# Autodesk Inventor assembly: s-assy-sorter
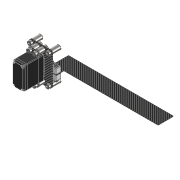
[picture p0: Inventor's stored thumbnail of the model, 180x180]
Saved by Autodesk Inventor 2022 (Build 260153000, 153)
## iProperties
Created: 2021-08-27
Part Number: s-assy-sorter
Document SubType Name: Assembly
Designer: Yuta Kage
Author: Yuta Kage
## Documents named in this file (9)
- C:\Users\yuta0\Documents\GitHub\catchrobo_hardware\assy-shooter\s-assy-sorter.iam
- C:\Users\yuta0\Documents\GitHub\catchrobo_hardware\assy-shooter\s-assy-shooter_motor.iam
- C:\Users\yuta0\Documents\GitHub\catchrobo_hardware\assy-shooter\s_base3.ipt
- C:\Users\yuta0\Documents\GitHub\catchrobo_hardware\assy-shooter\CB3-25.ipt
- C:\Users\yuta0\Documents\GitHub\catchrobo_hardware\assy-shooter\s_carbon_plate2.ipt
- C:\Users\yuta0\Documents\GitHub\catchrobo_hardware\assy-robot\CBSTNR3-12.ipt
- C:\Users\yuta0\Documents\GitHub\catchrobo_hardware\assy-robot\LBNR3.ipt
- C:\Users\yuta0\Documents\GitHub\catchrobo_hardware\assy-robot\ARF-415.ipt
- C:\Users\yuta0\Documents\GitHub\catchrobo_hardware\assy-robot\CB4-6.ipt
## Components (19 placed, 8 different names)
1. s-assy-shooter_motor:1 [sub-assembly] — メイト:6, メイト:7, メイト:12, メイト:13, メイト:14, メイト:15, メイト:16, メイト:17, メイト:18, メイト:19, メイト:20, メイト:21, メイト:22, メイト:23, メイト:24, メイト:25, メイト:26, メイト:27
2. s_base3:1 — メイト:6, メイト:7, メイト:8, メイト:9, メイト:11
3. s_carbon_plate2:1 — 角度:2
4. ARF-415:1 — メイト:12, メイト:18
5. ARF-415:2 — メイト:13, メイト:19
6. ARF-415:3 — メイト:14, メイト:17
7. ARF-415:4 — メイト:15, メイト:16
8. CB4-6:1 — メイト:23, メイト:24
9. CB4-6:2 — メイト:22, メイト:25
10. CB4-6:3 — メイト:21, メイト:26
11. CB4-6:4 — メイト:20, メイト:27
12. CBSTNR3-12:1 — メイト:8, メイト:9
13. CBSTNR3-12:2
14. CBSTNR3-12:3
15. CBSTNR3-12:4
16. CB3-25:1 — メイト:10
17. LBNR3:1 — メイト:10, メイト:11
18. CB3-25:2
19. LBNR3:2
## Component patterns: (4 elements, first: CBSTNR3-12:1), (2 elements, first: CB3-25:1 + LBNR3:1)
## Relationships (28: Mate 27, Angle 1)
- [Mate]: s_base3:1 ↔ s_carbon_plate2:1
- [Mate]: s_base3:1 ↔ s_carbon_plate2:1
- [Mate]: s_base3:1 ↔ s_carbon_plate2:1
- [Mate]: s_base3:1 ↔ CB3-25:1
- [Mate]: s_base3:1 ↔ CB3-25:1
- メイト:6 [Mate]: s-assy-shooter_motor:1 ↔ s_base3:1
- メイト:7 [Mate]: s-assy-shooter_motor:1 ↔ s_base3:1
- 角度:2 [Angle] (180 deg): s_carbon_plate2:1
- メイト:8 [Mate]: s_base3:1 ↔ CBSTNR3-12:1
- メイト:9 [Mate]: s_base3:1 ↔ CBSTNR3-12:1
- メイト:10 [Mate]: CB3-25:1 ↔ LBNR3:1
- メイト:11 [Mate]: s_base3:1 ↔ LBNR3:1
- メイト:12 [Mate]: s-assy-shooter_motor:1 ↔ ARF-415:1
- メイト:13 [Mate]: s-assy-shooter_motor:1 ↔ ARF-415:2
- メイト:14 [Mate]: s-assy-shooter_motor:1 ↔ ARF-415:3
- メイト:15 [Mate]: s-assy-shooter_motor:1 ↔ ARF-415:4
- メイト:16 [Mate]: s-assy-shooter_motor:1 ↔ ARF-415:4
- メイト:17 [Mate]: s-assy-shooter_motor:1 ↔ ARF-415:3
- メイト:18 [Mate]: s-assy-shooter_motor:1 ↔ ARF-415:1
- メイト:19 [Mate]: s-assy-shooter_motor:1 ↔ ARF-415:2
- メイト:20 [Mate]: s-assy-shooter_motor:1 ↔ CB4-6:4
- メイト:21 [Mate]: s-assy-shooter_motor:1 ↔ CB4-6:3
- メイト:22 [Mate]: s-assy-shooter_motor:1 ↔ CB4-6:2
- メイト:23 [Mate]: s-assy-shooter_motor:1 ↔ CB4-6:1
- メイト:24 [Mate]: s-assy-shooter_motor:1 ↔ CB4-6:1
- メイト:25 [Mate]: s-assy-shooter_motor:1 ↔ CB4-6:2
- メイト:26 [Mate]: s-assy-shooter_motor:1 ↔ CB4-6:3
- メイト:27 [Mate]: s-assy-shooter_motor:1 ↔ CB4-6:4
## Named parameters: d59_d15 = 0 mm, d62_d34 = 0 mm, d63_d35 = 0 mm, d64_d36 = 0 mm, d65_d37 = 0 mm
